# Autodesk Inventor assembly: Engranajes
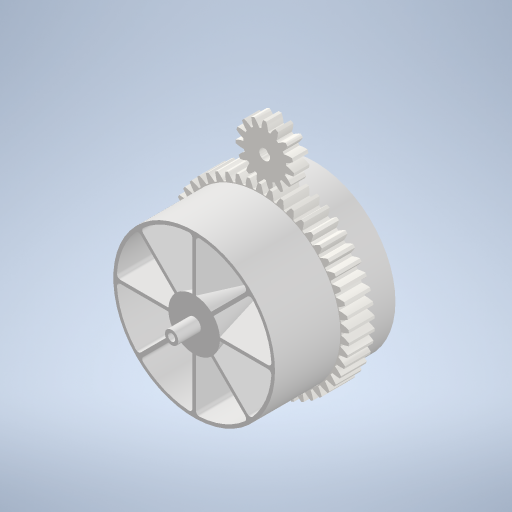
[picture p0: Inventor's stored thumbnail of the model, 512x512]
Saved by Autodesk Inventor 2024 (Build 280153000, 153)
## iProperties
Created: 2024-07-18
Part Number: Engranajes
Document SubType Name: Assembly
Designer: sergi
Author: sergi
## Documents named in this file (3)
- C:\Users\sergi\OneDrive\Escritorio\proyectos\ComederoV6\Engranajes.iam
- C:\Users\sergi\OneDrive\Escritorio\proyectos\ComederoV6\Dosificador.ipt
- C:\Users\sergi\OneDrive\Escritorio\proyectos\ComederoV6\Engranajes\Design Accelerator\Engranajes rectos2.iam
## Components (2 placed, 2 different names)
1. Dosificador:1 — Nivelación:1, Coincidencia:1
2. Engranajes rectos:1 [sub-assembly] — Nivelación:1, Coincidencia:1
## Relationships (2: Flush 1, Mate 1)
- Nivelación:1 [Flush] (38 mm): Dosificador:1 ↔ Engranajes rectos:1
- Coincidencia:1 [Mate]: Dosificador:1 ↔ Engranajes rectos:1
